# Autodesk Inventor assembly: Extree
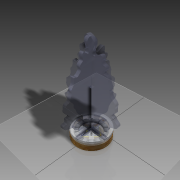
[picture p0: Inventor's stored thumbnail of the model, 180x180]
Saved by Autodesk Inventor 2014 (Build 180170000, 170)
## iProperties
Created: 2013-12-17
Part Number: Extree
Document SubType Name: Assembly
Designer: blacki
Author: blacki
## Documents named in this file (10)
- E:\Projects\Extree\00_Mechanical\Extree.iam
- E:\Projects\Extree\00_Mechanical\Side00.ipt
- E:\Projects\Extree\00_Mechanical\AdafruitNeoPixelRing16x.ipt
- E:\Projects\Extree\00_Mechanical\Side01.ipt
- E:\Projects\Extree\00_Mechanical\ArduinoProMini.ipt
- E:\Projects\Extree\00_Mechanical\TransparentTop.ipt
- E:\Projects\Extree\00_Mechanical\TreeHolder.ipt
- E:\Projects\Extree\00_Mechanical\ElectronicsHolder.ipt
- E:\Projects\Extree\00_Mechanical\LedHolder.ipt
- E:\Projects\Extree\00_Mechanical\BottomHolder.ipt
## Components (9 placed, 9 different names)
1. Side00:1 — Mate:1, Mate:3, Flush:1, Mate:6, Angle:1
2. AdafruitNeoPixelRing16x:1 — Mate:2, Mate:7, Mate:8
3. Side01:1 — Mate:1, Mate:4, Mate:5, Flush:2
4. ArduinoProMini:1 — Mate:2, Tangent:1, Tangent:2, Mate:12
5. TransparentTop:1 — Mate:3, Mate:4, Flush:1, Mate:5, Flush:2, Mate:6, Mate:7, Mate:8, Flush:3, Mate:9, Mate:10, Mate:14
6. TreeHolder:1 — Flush:3, Mate:9, Angle:1, Mate:13
7. ElectronicsHolder:1 — Mate:10, Tangent:1, Tangent:2, Mate:12, Flush:4, Flush:5, Flush:6, Mate:15
8. LedHolder:1 — Flush:4, Mate:13, Flush:5, Mate:14
9. BottomHolder:1 — Flush:6, Mate:15
## Relationships (23: Mate 14, Flush 6, Tangent 2, Angle 1)
- Mate:1: Side00:1 ↔ Side01:1
- Mate:2: AdafruitNeoPixelRing16x:1 ↔ ArduinoProMini:1
- Mate:3: Side00:1 ↔ TransparentTop:1
- Mate:4: Side01:1 ↔ TransparentTop:1
- Flush:1: Side00:1 ↔ TransparentTop:1
- Mate:5: Side01:1 ↔ TransparentTop:1
- Flush:2: Side01:1 ↔ TransparentTop:1
- Mate:6: Side00:1 ↔ TransparentTop:1
- Mate:7: AdafruitNeoPixelRing16x:1 ↔ TransparentTop:1
- Mate:8: AdafruitNeoPixelRing16x:1 ↔ TransparentTop:1
- Flush:3: TransparentTop:1 ↔ TreeHolder:1
- Mate:9: TransparentTop:1 ↔ TreeHolder:1
- Angle:1 (45 deg): Side00:1 ↔ TreeHolder:1
- Mate:10: TransparentTop:1 ↔ ElectronicsHolder:1
- Tangent:1 (1 mm): ArduinoProMini:1 ↔ ElectronicsHolder:1
- Tangent:2 (1 mm): ArduinoProMini:1 ↔ ElectronicsHolder:1
- Mate:12: ArduinoProMini:1 ↔ ElectronicsHolder:1
- Flush:4: ElectronicsHolder:1 ↔ LedHolder:1
- Mate:13: TreeHolder:1 ↔ LedHolder:1
- Flush:5: ElectronicsHolder:1 ↔ LedHolder:1
- Mate:14: TransparentTop:1 ↔ LedHolder:1
- Flush:6: ElectronicsHolder:1 ↔ BottomHolder:1
- Mate:15: ElectronicsHolder:1 ↔ BottomHolder:1
